# Autodesk Inventor assembly: New mounting
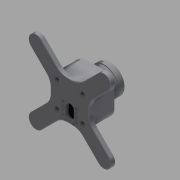
[picture p0: Inventor's stored thumbnail of the model, 180x180]
Saved by Autodesk Inventor 2017 (Build 210142000, 142)
## iProperties
Created: 2017-06-05
Part Number: New mounting
Document SubType Name: Assembly
Designer: Ali
Author: Ali
## Documents named in this file (7)
- F:\Documents\GitHub\EvoArm\Design\Experimental\New mounting.iam
- F:\Documents\GitHub\EvoArm\Design\Experimental\Arm - mounting v2.ipt
- F:\Documents\GitHub\EvoArm\Design\Parts\ax12_box.ipt
- F:\Documents\GitHub\EvoArm\Design\Parts\ax12_wheel.ipt
- F:\Documents\GitHub\EvoArm\Design\Experimental\Arm - slew column A.ipt
- F:\Documents\GitHub\EvoArm\Design\Experimental\Arm - slew column B.ipt
- F:\Documents\GitHub\EvoArm\Design\Experimental\Arm - slew column C.ipt
## Components (6 placed, 6 different names)
1. Arm - mounting v2:1 — Rigid:1
2. ax12_box:1 — Rotational:1, Rigid:1
3. ax12_wheel:1 — Rotational:1, Rigid:2
4. Arm - slew column A:1 — Rigid:2, Rigid:3
5. Arm - slew column B:1 — Rigid:3, Rigid:4
6. Arm - slew column C:1 — Rigid:4
## Relationships (5: WeldJoint 4, RevoluteJoint 1)
- Rotational:1 [RevoluteJoint]: ax12_box:1 ↔ ax12_wheel:1
- Rigid:1 [WeldJoint]: Arm - mounting v2:1 ↔ ax12_box:1
- Rigid:2 [WeldJoint]: ax12_wheel:1 ↔ Arm - slew column A:1
- Rigid:3 [WeldJoint]: Arm - slew column A:1 ↔ Arm - slew column B:1
- Rigid:4 [WeldJoint]: Arm - slew column B:1 ↔ Arm - slew column C:1
